# Autodesk Inventor assembly: Gripper2
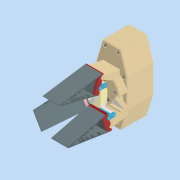
[picture p0: Inventor's stored thumbnail of the model, 180x180]
Saved by Autodesk Inventor 2020.3 (Build 243373000, 373)
## iProperties
Created: 2020-03-10
Part Number: Gripper2
Document SubType Name: Assembly
Designer: JochenAlt
Author: JochenAlt
## Documents named in this file (22)
- D:\Projects\MiniBot\CAD\gripper\Gripper.iam
- D:\Projects\MiniBot\CAD\gripper\Centre.ipt
- D:\Projects\MiniBot\CAD\gripper\GripperCompensator.ipt
- D:\Projects\MiniBot\CAD\gripper\Lever.ipt
- D:\Projects\MiniBot\CAD\gripper\Finger.iam
- D:\Projects\MiniBot\CAD\gripper\GripTypeLever.ipt
- D:\Projects\MiniBot\CAD\extern\Herkulex\Herkulex DRS-020x.ipt
- D:\Projects\MiniBot\CAD\gripper\Gripper\Konstruktions-Assistent\Schneckenräder1.iam
- D:\Projects\MiniBot\CAD\gripper\Base\Konstruktions-Assistent\Schnecke1.ipt
- D:\Projects\MiniBot\CAD\gripper\Base.ipt
- D:\Projects\MiniBot\CAD\WristGear\Konstruktions-Assistent\Stirnräder2.iam
- D:\Projects\MiniBot\CAD\extern\bearings\4x7x2.5\W 627_4-2ZS.iam
- D:\Projects\MiniBot\CAD\extern\bearings\3x7x2\W 618_3.iam
- D:\Projects\MiniBot\CAD\extern\bearings\5x9x3\W 637_5 X-2Z.iam
- C:\Users\JochenAlt\Documents\Inventor\Content Center Files\R2020\de-DE\DIN 125-1  A\DIN 125 - A 2,2.ipt
- C:\Users\JochenAlt\Documents\Inventor\Content Center Files\R2020\de-DE\DIN 912\DIN 912 - M2 x 0,4 x 12 x 11.ipt
- C:\Users\JochenAlt\Documents\Inventor\Content Center Files\R2020\de-DE\DIN 912\DIN 912 - M2 x 0,4 x 16 x 15.ipt
- C:\Users\JochenAlt\Documents\Inventor\Content Center Files\R2020\de-DE\DIN 912\DIN 912 - M2 x 0,4 x 10 x 9.ipt
- C:\Users\JochenAlt\Documents\Inventor\Content Center Files\R2020\de-DE\DIN 934\DIN 934 - M2 x 0,4.ipt
- C:\Users\JochenAlt\Documents\Inventor\Content Center Files\R2020\de-DE\DIN 912\DIN 912 - M2 x 0,4 x 20 x 19.ipt
- C:\Users\JochenAlt\Documents\Inventor\Content Center Files\R2020\de-DE\DIN 912\DIN 912 - M2,5 x 0,45 x 12 x 10,875.ipt
- C:\Users\JochenAlt\Documents\Inventor\Content Center Files\R2020\de-DE\DIN 912\DIN 912 - M2,5 x 0,45 x 16 x 14,875.ipt
## Components (46 placed, 21 different names)
1. GripperCompensator:1 — Drehung:1, Fluchtend:7, Passend:59, Fluchtend:14, Fluchtend:23, Passend:101
2. GripperCompensator:2 — Drehung:1, Fluchtend:7, Fluchtend:14, Passend:65, Passend:93, Fluchtend:23, Passend:102
3. CentreGripLever:11 — Passend:54, Passend:59, Fluchtend:13
4. CentreGripLever:12 — Passend:55, Fluchtend:11, Passend:148
5. CentreGripLever:13 — Passend:56, Passend:65, Fluchtend:29
6. Finger:4 [sub-assembly] — Passend:54, Fluchtend:13, Passend:178, Fluchtend:28
7. Finger:5 [sub-assembly] — Passend:55, Fluchtend:11, Passend:108, Passend:110, Fluchtend:26
8. Finger:6 [sub-assembly] — Passend:56, Passend:179, Fluchtend:29, Fluchtend:30
9. GripTypeLever:1 — Fluchtend:27, Passend:178, Fluchtend:28, Winkel:4, Passend:208
10. GripTypeLever:2 — Fluchtend:27, Passend:179, Fluchtend:30, Winkel:5, Passend:191, Fluchtend:31
11. Herkulex DRS-0201:1 — Passend:145, Passend:188, Passend:189
12. Herkulex DRS-0201:2 — Passend:187
13. Centre:1 — Passend:93, Passend:101, Passend:102, Passend:147, Passend:148
14. Schneckenräder:1 [sub-assembly]
15. Schnecke:1 — Passend:139, Passend:141
16. Base:1 — Passend:108, Passend:110, Fluchtend:26, Passend:146, Winkel:4, Winkel:5, Passend:182, Passend:183, Passend:187, Passend:189, Passend:191, Passend:192, Passend:193, Passend:194, Passend:195, Passend:198, Passend:199, Passend:200, Passend:201, Einfügen:1, Einfügen:2, Einfügen:3, Einfügen:4, Einfügen:5, Einfügen:6, Einfügen:7, Einfügen:8, Einfügen:9, Einfügen:10, Einfügen:12, Einfügen:13, Einfügen:14, Einfügen:15, Einfügen:16, Einfügen:17, Einfügen:18, Passend:206, Passend:207, Fluchtend:31, Passend:208
17. Stirnräder:1 [sub-assembly] — Passend:130, Passend:131, Passend:141, Passend:144, Passend:145, Passend:146, Passend:147, Passend:188
18. W 627_4-2ZS:1 [sub-assembly] — Passend:130, Passend:144, Passend:183
19. W 627_4-2ZS:2 [sub-assembly] — Passend:131, Passend:139, Passend:182
20. W 618_3:1 [sub-assembly] — Passend:192, Passend:206, Einfügen:19
21. W 618_3:2 [sub-assembly] — Passend:195, Passend:198
22. W 618_3:3 [sub-assembly] — Passend:193, Passend:207, Einfügen:20
23. W 618_3:4 [sub-assembly] — Passend:194, Passend:199
24. W 637_5 X-2Z:1 [sub-assembly] — Passend:200, Passend:201
25. DIN 912 - ersetzt durch DIN EN ISO 4762 M2 x 10:1 — Einfügen:1
26. DIN 912 - ersetzt durch DIN EN ISO 4762 M2 x 10:2 — Einfügen:2
27. DIN 912 - ersetzt durch DIN EN ISO 4762 M2 x 10:3 — Einfügen:3
28. DIN 912 - ersetzt durch DIN EN ISO 4762 M2 x 10:4 — Einfügen:4
29. DIN 912 - ersetzt durch DIN EN ISO 4762 M2 x 16:1 — Einfügen:5, Passend:204, Passend:205
30. DIN 912 - ersetzt durch DIN EN ISO 4762 M2 x 16:2 — Einfügen:6, Passend:202, Passend:203
31. DIN 912 - ersetzt durch DIN EN ISO 4762 M2 x 10:7 — Einfügen:7
32. DIN 912 - ersetzt durch DIN EN ISO 4762 M2 x 10:8 — Einfügen:8
33. DIN 912 - ersetzt durch DIN EN ISO 4762 M2 x 10:9 — Einfügen:9
34. DIN 125-1 A A 2,2:1 — Einfügen:10, Einfügen:11
35. DIN 912 - ersetzt durch DIN EN ISO 4762 M2 x 12:1 — Einfügen:11
36. DIN 934 - ersetzt durch DIN EN 24032/28673/28674 M2:1 — Passend:202, Passend:203
37. DIN 934 - ersetzt durch DIN EN 24032/28673/28674 M2:2 — Passend:204, Passend:205
38. DIN 912 - ersetzt durch DIN EN ISO 4762 M2 x 20:1 — Einfügen:12
39. DIN 912 - ersetzt durch DIN EN ISO 4762 M2 x 20:2 — Einfügen:13
40. DIN 912 - ersetzt durch DIN EN ISO 4762 M2 x 20:3 — Einfügen:14
41. DIN 912 - ersetzt durch DIN EN ISO 4762 M2 x 10:10 — Einfügen:15
42. DIN 912 - ersetzt durch DIN EN ISO 4762 M2 x 10:11 — Einfügen:16
43. DIN 912 - ersetzt durch DIN EN ISO 4762 M2 x 10:12 — Einfügen:17
44. DIN 912 - ersetzt durch DIN EN ISO 4762 M2 x 10:13 — Einfügen:18
45. DIN 912 - ersetzt durch DIN EN ISO 4762 M2,5 x 12:1 — Einfügen:19
46. DIN 912 - ersetzt durch DIN EN ISO 4762 M2,5 x 16:1 — Einfügen:20
## Relationships (76: Mate 42, Insert 20, Flush 11, Angle 2, RelateRotation 1)
- Drehung:1 [RelateRotation] (1 ul): GripperCompensator:1 ↔ GripperCompensator:2
- Fluchtend:7 [Flush]: GripperCompensator:1 ↔ GripperCompensator:2
- Passend:54 [Mate]: CentreGripLever:11 ↔ Finger:4
- Passend:55 [Mate]: CentreGripLever:12 ↔ Finger:5
- Passend:56 [Mate]: CentreGripLever:13 ↔ Finger:6
- Passend:59 [Mate]: GripperCompensator:1 ↔ CentreGripLever:11
- Fluchtend:11 [Flush]: CentreGripLever:12 ↔ Finger:5
- Fluchtend:13 [Flush]: CentreGripLever:11 ↔ Finger:4
- Fluchtend:14 [Flush]: GripperCompensator:1 ↔ GripperCompensator:2
- Passend:65 [Mate]: GripperCompensator:2 ↔ CentreGripLever:13
- Passend:93 [Mate] (0.25 mm): GripperCompensator:2 ↔ Centre:1
- Fluchtend:23 [Flush]: GripperCompensator:1 ↔ GripperCompensator:2
- Passend:101 [Mate]: GripperCompensator:1 ↔ Centre:1
- Passend:102 [Mate]: GripperCompensator:2 ↔ Centre:1
- Passend:108 [Mate]: Finger:5 ↔ Base:1
- Passend:110 [Mate]: Finger:5 ↔ Base:1
- Fluchtend:26 [Flush]: Finger:5 ↔ Base:1
- Passend:130 [Mate]: Stirnräder:1 ↔ W 627_4-2ZS:1
- Passend:131 [Mate]: Stirnräder:1 ↔ W 627_4-2ZS:2
- Passend:139 [Mate]: Schnecke:1 ↔ W 627_4-2ZS:2
- Passend:141 [Mate]: Schnecke:1 ↔ Stirnräder:1
- Passend:144 [Mate]: Stirnräder:1 ↔ W 627_4-2ZS:1
- Passend:145 [Mate]: Herkulex DRS-0201:1 ↔ Stirnräder:1
- Passend:146 [Mate]: Base:1 ↔ Stirnräder:1
- Passend:147 [Mate]: Centre:1 ↔ Stirnräder:1
- Passend:148 [Mate]: CentreGripLever:12 ↔ Centre:1
- Fluchtend:27 [Flush]: GripTypeLever:1 ↔ GripTypeLever:2
- Passend:178 [Mate]: Finger:4 ↔ GripTypeLever:1
- Fluchtend:28 [Flush]: Finger:4 ↔ GripTypeLever:1
- Passend:179 [Mate]: Finger:6 ↔ GripTypeLever:2
- Fluchtend:29 [Flush]: CentreGripLever:13 ↔ Finger:6
- Fluchtend:30 [Flush]: Finger:6 ↔ GripTypeLever:2
- Winkel:4 [Angle] (120 deg): GripTypeLever:1 ↔ Base:1
- Winkel:5 [Angle] (180 deg): GripTypeLever:2 ↔ Base:1
- Passend:182 [Mate]: Base:1 ↔ W 627_4-2ZS:2
- Passend:183 [Mate]: Base:1 ↔ W 627_4-2ZS:1
- Passend:187 [Mate]: Herkulex DRS-0201:2 ↔ Base:1
- Passend:188 [Mate]: Herkulex DRS-0201:1 ↔ Stirnräder:1
- Passend:189 [Mate]: Herkulex DRS-0201:1 ↔ Base:1
- Passend:191 [Mate]: GripTypeLever:2 ↔ Base:1
- Passend:192 [Mate]: Base:1 ↔ W 618_3:1
- Passend:193 [Mate]: Base:1 ↔ W 618_3:3
- Passend:194 [Mate]: Base:1 ↔ W 618_3:4
- Passend:195 [Mate]: Base:1 ↔ W 618_3:2
- Passend:198 [Mate]: Base:1 ↔ W 618_3:2
- Passend:199 [Mate]: Base:1 ↔ W 618_3:4
- Passend:200 [Mate]: Base:1 ↔ W 637_5 X-2Z:1
- Passend:201 [Mate]: Base:1 ↔ W 637_5 X-2Z:1
- Einfügen:1 [Insert]: Base:1 ↔ DIN 912 - ersetzt durch DIN EN ISO 4762 M2 x 10:1
- Einfügen:2 [Insert]: Base:1 ↔ DIN 912 - ersetzt durch DIN EN ISO 4762 M2 x 10:2
- Einfügen:3 [Insert]: Base:1 ↔ DIN 912 - ersetzt durch DIN EN ISO 4762 M2 x 10:3
- Einfügen:4 [Insert]: Base:1 ↔ DIN 912 - ersetzt durch DIN EN ISO 4762 M2 x 10:4
- Einfügen:5 [Insert]: Base:1 ↔ DIN 912 - ersetzt durch DIN EN ISO 4762 M2 x 16:1
- Einfügen:6 [Insert]: Base:1 ↔ DIN 912 - ersetzt durch DIN EN ISO 4762 M2 x 16:2
- Einfügen:7 [Insert]: Base:1 ↔ DIN 912 - ersetzt durch DIN EN ISO 4762 M2 x 10:7
- Einfügen:8 [Insert]: Base:1 ↔ DIN 912 - ersetzt durch DIN EN ISO 4762 M2 x 10:8
- Einfügen:9 [Insert]: Base:1 ↔ DIN 912 - ersetzt durch DIN EN ISO 4762 M2 x 10:9
- Einfügen:10 [Insert]: Base:1 ↔ DIN 125-1 A A 2,2:1
- Einfügen:11 [Insert]: DIN 125-1 A A 2,2:1 ↔ DIN 912 - ersetzt durch DIN EN ISO 4762 M2 x 12:1
- Passend:202 [Mate]: DIN 912 - ersetzt durch DIN EN ISO 4762 M2 x 16:2 ↔ DIN 934 - ersetzt durch DIN EN 24032/28673/28674 M2:1
- Passend:203 [Mate]: DIN 912 - ersetzt durch DIN EN ISO 4762 M2 x 16:2 ↔ DIN 934 - ersetzt durch DIN EN 24032/28673/28674 M2:1
- Passend:204 [Mate]: DIN 912 - ersetzt durch DIN EN ISO 4762 M2 x 16:1 ↔ DIN 934 - ersetzt durch DIN EN 24032/28673/28674 M2:2
- Passend:205 [Mate]: DIN 912 - ersetzt durch DIN EN ISO 4762 M2 x 16:1 ↔ DIN 934 - ersetzt durch DIN EN 24032/28673/28674 M2:2
- Einfügen:12 [Insert]: Base:1 ↔ DIN 912 - ersetzt durch DIN EN ISO 4762 M2 x 20:1
- Einfügen:13 [Insert]: Base:1 ↔ DIN 912 - ersetzt durch DIN EN ISO 4762 M2 x 20:2
- Einfügen:14 [Insert]: Base:1 ↔ DIN 912 - ersetzt durch DIN EN ISO 4762 M2 x 20:3
- Einfügen:15 [Insert]: Base:1 ↔ DIN 912 - ersetzt durch DIN EN ISO 4762 M2 x 10:10
- Einfügen:16 [Insert]: Base:1 ↔ DIN 912 - ersetzt durch DIN EN ISO 4762 M2 x 10:11
- Einfügen:17 [Insert]: Base:1 ↔ DIN 912 - ersetzt durch DIN EN ISO 4762 M2 x 10:12
- Einfügen:18 [Insert]: Base:1 ↔ DIN 912 - ersetzt durch DIN EN ISO 4762 M2 x 10:13
- Passend:206 [Mate]: Base:1 ↔ W 618_3:1
- Passend:207 [Mate]: Base:1 ↔ W 618_3:3
- Einfügen:19 [Insert]: W 618_3:1 ↔ DIN 912 - ersetzt durch DIN EN ISO 4762 M2,5 x 12:1
- Einfügen:20 [Insert]: W 618_3:3 ↔ DIN 912 - ersetzt durch DIN EN ISO 4762 M2,5 x 16:1
- Fluchtend:31 [Flush]: GripTypeLever:2 ↔ Base:1
- Passend:208 [Mate]: GripTypeLever:1 ↔ Base:1
